# Autodesk Inventor assembly: kosi_v2
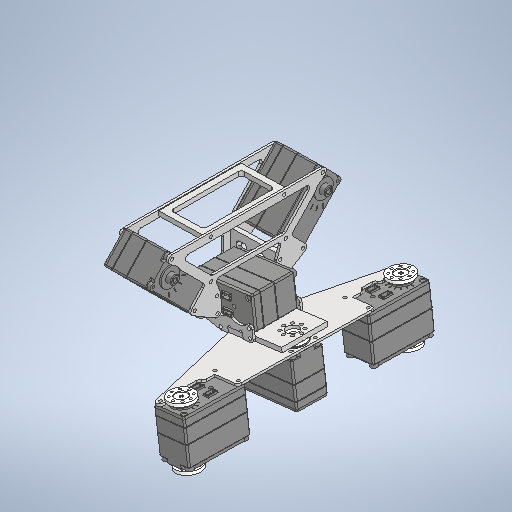
[picture p0: Inventor's stored thumbnail of the model, 512x512]
Saved by Autodesk Inventor 2025.1 (Build 291241000, 241)
## iProperties
Created: 2024-08-31
Part Number: kosi_v2
Document SubType Name: Assembly
Designer: right
Author: right
## Documents named in this file (12)
- C:\Users\right\Documents\Inventor\Vixen\kosi_v2.iam
- C:\Users\right\Documents\Inventor\Vixen\KRS2500_scale.ipt
- C:\Users\right\Documents\Inventor\Vixen\02157_SmallDiameterHornB.ipt
- C:\Users\right\Documents\Inventor\Vixen\02159_SmallFreeHornC\02159_SmallFreeHornC.ipt
- C:\Users\right\Documents\Inventor\Vixen\piti_mata.ipt
- C:\Users\right\Documents\Inventor\Vixen\kosipich.ipt
- C:\Users\right\Documents\Inventor\Vixen\senakamata.ipt
- C:\Users\right\Documents\Inventor\Vixen\kosiyosetuzoku.ipt
- C:\Users\right\Documents\Inventor\Vixen\kosiyo.ipt
- C:\Users\right\Documents\Inventor\Vixen\kosinosita.ipt
- C:\Users\right\Documents\Inventor\Vixen\jouhansinsita.ipt
- C:\Users\right\Documents\Inventor\Vixen\jouhansin_sita.ipt
## Components (23 placed, 11 different names)
1. KRS2500_scale:1 — 挿入:17, 挿入:42, 挿入:43
2. KRS2500_scale:2 — 挿入:40
3. 02159_SmallFreeHornC:1 — 挿入:15, 挿入:35, 挿入:36
4. KRS2500_scale:4 — 挿入:15, 挿入:30, 角度:2, 挿入:45, 挿入:46, 挿入:47, 挿入:48
5. piti_mata:1 — 挿入:17, 挿入:31, 挿入:32, 挿入:43, 挿入:59, 挿入:60
6. 02157_SmallDiameterHornB:2 — 挿入:30, 挿入:33, 挿入:34
7. kosipich:1 — 挿入:31, 挿入:32, 挿入:33, 挿入:34
8. kosipich:2 — 挿入:35, 挿入:36, フラッシュ:1, 挿入:41
9. senakamata:1 — フラッシュ:1, 挿入:40, 挿入:41, 挿入:42, フラッシュ:6, 挿入:57, 挿入:58
10. KRS2500_scale:5 — 挿入:44, 角度:2, フラッシュ:2, 角度:3, フラッシュ:3, メイト:1, メイト:2, 角度:4, フラッシュ:4, フラッシュ:5, フラッシュ:8
11. 02157_SmallDiameterHornB:3 — 挿入:44, 挿入:51, 挿入:52
12. kosiyosetuzoku:1 — 挿入:45, 挿入:46, 挿入:50
13. kosiyosetuzoku:2 — 挿入:47, 挿入:48, 挿入:49
14. kosiyo:1 — 挿入:49, 挿入:50, 挿入:51, 挿入:52, フラッシュ:7
15. 02159_SmallFreeHornC:2
16. KRS2500_scale:6 — フラッシュ:2, 角度:3, フラッシュ:3, メイト:1
17. 02157_SmallDiameterHornB:4
18. 02159_SmallFreeHornC:3
19. KRS2500_scale:7 — メイト:2, 角度:4, フラッシュ:4, フラッシュ:5
20. 02157_SmallDiameterHornB:5
21. kosinosita:1 — フラッシュ:6, 挿入:57, 挿入:58, 挿入:59, 挿入:60
22. jouhansinsita:1 — フラッシュ:7
23. jouhansin_sita:1 — フラッシュ:8
## Relationships (43: Insert 30, Flush 8, Angle 3, Mate 2)
- 挿入:15 [Insert]: 02159_SmallFreeHornC:1 ↔ KRS2500_scale:4
- 挿入:17 [Insert]: KRS2500_scale:1 ↔ piti_mata:1
- 挿入:30 [Insert]: KRS2500_scale:4 ↔ 02157_SmallDiameterHornB:2
- 挿入:31 [Insert]: piti_mata:1 ↔ kosipich:1
- 挿入:32 [Insert]: piti_mata:1 ↔ kosipich:1
- 挿入:33 [Insert]: 02157_SmallDiameterHornB:2 ↔ kosipich:1
- 挿入:34 [Insert]: 02157_SmallDiameterHornB:2 ↔ kosipich:1
- 挿入:35 [Insert]: 02159_SmallFreeHornC:1 ↔ kosipich:2
- 挿入:36 [Insert]: 02159_SmallFreeHornC:1 ↔ kosipich:2
- フラッシュ:1 [Flush]: kosipich:2 ↔ senakamata:1
- 挿入:40 [Insert]: KRS2500_scale:2 ↔ senakamata:1
- 挿入:41 [Insert]: kosipich:2 ↔ senakamata:1
- 挿入:42 [Insert]: KRS2500_scale:1 ↔ senakamata:1
- 挿入:43 [Insert]: KRS2500_scale:1 ↔ piti_mata:1
- 挿入:44 [Insert]: KRS2500_scale:5 ↔ 02157_SmallDiameterHornB:3
- 角度:2 [Angle] (0 deg): KRS2500_scale:4 ↔ KRS2500_scale:5
- 挿入:45 [Insert]: KRS2500_scale:4 ↔ kosiyosetuzoku:1
- 挿入:46 [Insert]: KRS2500_scale:4 ↔ kosiyosetuzoku:1
- 挿入:47 [Insert]: KRS2500_scale:4 ↔ kosiyosetuzoku:2
- 挿入:48 [Insert]: KRS2500_scale:4 ↔ kosiyosetuzoku:2
- 挿入:49 [Insert]: kosiyosetuzoku:2 ↔ kosiyo:1
- 挿入:50 [Insert]: kosiyosetuzoku:1 ↔ kosiyo:1
- 挿入:51 [Insert]: 02157_SmallDiameterHornB:3 ↔ kosiyo:1
- 挿入:52 [Insert]: 02157_SmallDiameterHornB:3 ↔ kosiyo:1
- [Insert]: 02159_SmallFreeHornC:2 ↔ KRS2500_scale:6
- [Insert]: KRS2500_scale:6 ↔ 02157_SmallDiameterHornB:4
- フラッシュ:2 [Flush]: KRS2500_scale:5 ↔ KRS2500_scale:6
- 角度:3 [Angle] (0 deg): KRS2500_scale:5 ↔ KRS2500_scale:6
- フラッシュ:3 [Flush]: KRS2500_scale:5 ↔ KRS2500_scale:6
- メイト:1 [Mate] (30 mm): KRS2500_scale:5 ↔ KRS2500_scale:6
- [Insert]: 02159_SmallFreeHornC:3 ↔ KRS2500_scale:7
- [Insert]: KRS2500_scale:7 ↔ 02157_SmallDiameterHornB:5
- メイト:2 [Mate] (30 mm): KRS2500_scale:5 ↔ KRS2500_scale:7
- 角度:4 [Angle] (180 deg): KRS2500_scale:5 ↔ KRS2500_scale:7
- フラッシュ:4 [Flush]: KRS2500_scale:5 ↔ KRS2500_scale:7
- フラッシュ:5 [Flush]: KRS2500_scale:5 ↔ KRS2500_scale:7
- フラッシュ:6 [Flush]: senakamata:1 ↔ kosinosita:1
- 挿入:57 [Insert]: senakamata:1 ↔ kosinosita:1
- 挿入:58 [Insert]: senakamata:1 ↔ kosinosita:1
- 挿入:59 [Insert]: piti_mata:1 ↔ kosinosita:1
- 挿入:60 [Insert]: piti_mata:1 ↔ kosinosita:1
- フラッシュ:7 [Flush]: kosiyo:1 ↔ jouhansinsita:1
- フラッシュ:8 [Flush]: KRS2500_scale:5 ↔ jouhansin_sita:1
## Named parameters: d78_d42 = 0 mm, d79_d26 = 0 mm, d84_d78_d42 = 0 mm, d85_d79_d26 = 0 mm
